# Autodesk Inventor assembly: Soyuz Launch Escape System
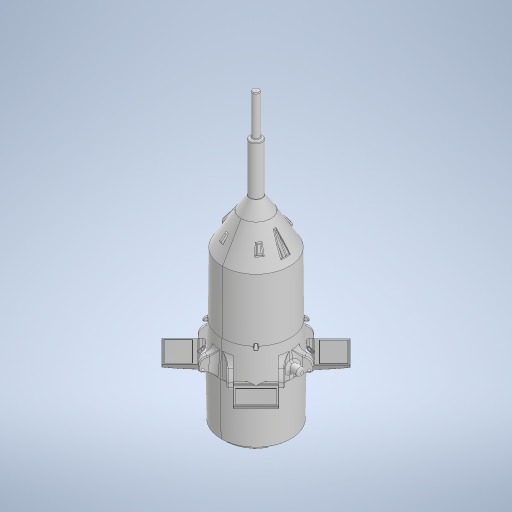
[picture p0: Inventor's stored thumbnail of the model, 512x512]
Saved by Autodesk Inventor 2023 (Build 270158030, 158C)
## iProperties
Created: 2023-01-09
Part Number: Soyuz Launch Escape System
Document SubType Name: Assembly
Designer: Imogen Heard
Author: Imogen Heard
## Documents named in this file (3)
- C:\Users\dheard\Documents\Inventor\Inventor_Projects\Soyuz Model\Soyuz Launch Escape System.iam
- C:\Users\dheard\Documents\Inventor\Inventor_Projects\Soyuz Model\Soyuz Fairing & Payload Bay Assembly Grid Fin Deploy.iam
- C:\Users\dheard\Documents\Inventor\Inventor_Projects\Soyuz Model\Escape Tower.ipt
## Components (3 placed, 2 different names)
1. Soyuz Fairing & Payload Bay Assembly Grid Fin Deploy:1 [sub-assembly] — Mate:1, Flush:1, Mate:2, Insert:1
2. Soyuz Fairing & Payload Bay Assembly Grid Fin Deploy:2 [sub-assembly] — Mate:1, Flush:1, Mate:2
3. Escape Tower:1 — Insert:1
## Relationships (4: Mate 2, Flush 1, Insert 1)
- Mate:1: Soyuz Fairing & Payload Bay Assembly Grid Fin Deploy:1 ↔ Soyuz Fairing & Payload Bay Assembly Grid Fin Deploy:2
- Flush:1: Soyuz Fairing & Payload Bay Assembly Grid Fin Deploy:1 ↔ Soyuz Fairing & Payload Bay Assembly Grid Fin Deploy:2
- Mate:2: Soyuz Fairing & Payload Bay Assembly Grid Fin Deploy:1 ↔ Soyuz Fairing & Payload Bay Assembly Grid Fin Deploy:2
- Insert:1: Soyuz Fairing & Payload Bay Assembly Grid Fin Deploy:1 ↔ Escape Tower:1
